# Autodesk Inventor assembly: Thruster Assembly
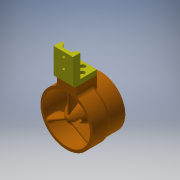
[picture p0: Inventor's stored thumbnail of the model, 180x180]
Saved by Autodesk Inventor 2017 (Build 210142000, 142)
## iProperties
Created: 2017-08-02
Part Number: Thruster Assembly
Document SubType Name: Assembly
Designer: Thein Lin Aung
Author: Thein Lin Aung
## Documents named in this file (5)
- C:\Users\Thein Lin Aung\Documents\Inventor\ROV Research\Thruster Assembly.iam
- C:\Users\Thein Lin Aung\Documents\Inventor\ROV Research\Brushless Motor.ipt
- C:\Users\Thein Lin Aung\Documents\Inventor\ROV Research\Propeller.ipt
- C:\Users\Thein Lin Aung\Documents\Inventor\ROV Research\Duct.ipt
- C:\Users\Thein Lin Aung\Documents\Inventor\ROV Research\Test Mount.ipt
## Components (4 placed, 4 different names)
1. Brushless Motor:1 — Mate:1, Mate:2, Mate:3, Flush:5, Mate:4, Angle:1
2. Propeller:1 — Mate:1, Mate:2, Angle:1
3. Duct:1 — Mate:3, Flush:5, Mate:4, Mate:5, Flush:6, Mate:6
4. Test Mount:1 — Mate:5, Flush:6, Mate:6
## Relationships (9: Mate 6, Flush 2, Angle 1)
- Mate:1: Brushless Motor:1 ↔ Propeller:1
- Mate:2: Brushless Motor:1 ↔ Propeller:1
- Mate:3: Brushless Motor:1 ↔ Duct:1
- Flush:5: Brushless Motor:1 ↔ Duct:1
- Mate:4: Brushless Motor:1 ↔ Duct:1
- Angle:1 (0 deg): Brushless Motor:1 ↔ Propeller:1
- Mate:5: Duct:1 ↔ Test Mount:1
- Flush:6: Duct:1 ↔ Test Mount:1
- Mate:6: Duct:1 ↔ Test Mount:1
